# Autodesk Inventor assembly: Trasmissione cinghie - Taglio
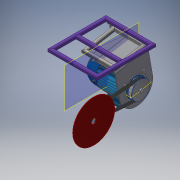
[picture p0: Inventor's stored thumbnail of the model, 180x180]
Saved by Autodesk Inventor 2018 (Build 220112000, 112)
## iProperties
Created: 2020-06-04
Part Number: Trasmissione cinghie - Taglio
Material: Generico
Document SubType Name: Assembly
Designer: Francesco
Author: Francesco
## Documents named in this file (8)
- C:\Users\Francesco\no-brim\Meccanica\Progetto Inventor no-brim\Assiemi\Trasmissione cinghie - Taglio.iam
- C:\Users\Francesco\no-brim\Meccanica\Progetto Inventor no-brim\Parti\Puleggia maggiore.ipt
- C:\Users\Francesco\no-brim\Meccanica\Progetto Inventor no-brim\Parti\Puleggia minore.ipt
- C:\Users\Francesco\no-brim\Meccanica\Progetto Inventor no-brim\Parti\Cinghia.ipt
- C:\Users\Francesco\no-brim\Meccanica\Progetto Inventor no-brim\Parti\Sega Circolare 300 mm.ipt
- C:\Users\Francesco\no-brim\Meccanica\Progetto Inventor no-brim\Parti\Motorredutor Bonfiglioli .iam
- C:\Users\Francesco\no-brim\Meccanica\Progetto Inventor no-brim\Parti\Lamiera supporto motore.ipt
- C:\Users\Francesco\no-brim\Meccanica\Progetto Inventor no-brim\Assiemi\Telaietto trasmissione - Taglio.iam
## Components (7 placed, 7 different names)
1. Puleggia maggiore:1 — Allineato:1, Coincidente:2, Coincidente:3, Coincidente:11, Angolo:1, Coincidente:15
2. Puleggia minore:1 — Allineato:1, Coincidente:1, Coincidente:4, Coincidente:10
3. Cinghia:1 — Coincidente:1, Coincidente:2, Coincidente:3
4. Sega Circolare 300 mm:1 — Coincidente:4, Coincidente:10
5. Lamiera supporto motore:1 — Coincidente:11, Angolo:1, Coincidente:13, Coincidente:14, Angolo:2, Coincidente:16, Allineato:6, Allineato:7
6. Motorredutor Bonfiglioli :1 [sub-assembly] — Coincidente:13, Coincidente:14, Angolo:2, Coincidente:15
7. Telaietto trasmissione:1 [sub-assembly] — Allineato:5, Coincidente:16, Allineato:6, Allineato:7
## Relationships (16: Mate 10, Flush 4, Angle 2)
- Allineato:1 [Flush]: Puleggia maggiore:1 ↔ Puleggia minore:1
- Coincidente:1 [Mate]: Puleggia minore:1 ↔ Cinghia:1
- Coincidente:2 [Mate]: Puleggia maggiore:1 ↔ Cinghia:1
- Coincidente:3 [Mate] (1.5 mm): Puleggia maggiore:1 ↔ Cinghia:1
- Coincidente:4 [Mate]: Puleggia minore:1 ↔ Sega Circolare 300 mm:1
- Coincidente:10 [Mate] (15 mm): Puleggia minore:1 ↔ Sega Circolare 300 mm:1
- Coincidente:11 [Mate]: Puleggia maggiore:1 ↔ Lamiera supporto motore:1
- Angolo:1 [Angle] (0 deg): Puleggia maggiore:1 ↔ Lamiera supporto motore:1
- Coincidente:13 [Mate]: Lamiera supporto motore:1 ↔ Motorredutor Bonfiglioli :1
- Coincidente:14 [Mate]: Lamiera supporto motore:1 ↔ Motorredutor Bonfiglioli :1
- Angolo:2 [Angle] (-90 deg): Lamiera supporto motore:1 ↔ Motorredutor Bonfiglioli :1
- Coincidente:15 [Mate]: Puleggia maggiore:1 ↔ Motorredutor Bonfiglioli :1
- Allineato:5 [Flush] (-150 mm): Telaietto trasmissione:1
- Coincidente:16 [Mate]: Lamiera supporto motore:1 ↔ Telaietto trasmissione:1
- Allineato:6 [Flush]: Lamiera supporto motore:1 ↔ Telaietto trasmissione:1
- Allineato:7 [Flush]: Lamiera supporto motore:1 ↔ Telaietto trasmissione:1
